# Autodesk Inventor assembly: crane-base-assembly
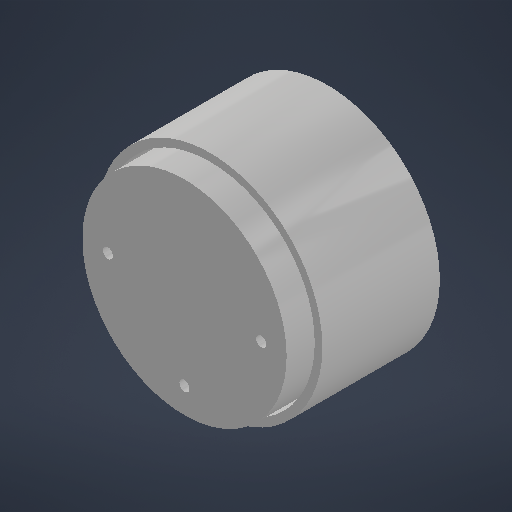
[picture p0: Inventor's stored thumbnail of the model, 512x512]
Saved by Autodesk Inventor 2026.2 (Build 302298010, 298A)
## iProperties
Created: 2026-02-25
Part Number: crane-base-assembly
Document SubType Name: Assembly
Designer: dm2166
Author: dm2166
## Documents named in this file (3)
- C:\Users\bobmi\OneDrive - Heriot-Watt University\Github\System-Project-G2\mechanical\crane-base-assembly.iam
- C:\Users\bobmi\OneDrive - Heriot-Watt University\Github\System-Project-G2\mechanical\rotating base head.ipt
- C:\Users\bobmi\OneDrive - Heriot-Watt University\Github\System-Project-G2\mechanical\rotating base bottom.ipt
## Components (2 placed, 2 different names)
1. rotating base head:1 — Insert:1
2. rotating base bottom:1 — Flush:1, Insert:1, Mate:1
## Relationships (3: Flush 1, Insert 1, Mate 1)
- Flush:1: rotating base bottom:1
- Insert:1: rotating base head:1 ↔ rotating base bottom:1
- Mate:1: rotating base bottom:1
